# Autodesk Inventor assembly: Linear Actuator 12inch
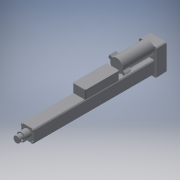
[picture p0: Inventor's stored thumbnail of the model, 180x180]
Saved by Autodesk Inventor 2016 (Build 200138000, 138)
## iProperties
Created: 2018-06-28
Part Number: Linear Actuator 12inch
Document SubType Name: Assembly
Designer: Kade
Author: Kade
## Documents named in this file (3)
- F:\Robotics\Off Season\Blannon\Linear Actuator\Linear Actuator 12inch.iam
- F:\Robotics\Off Season\Blannon\Linear Actuator\Linear Actuator Body.ipt
- F:\Robotics\Off Season\Blannon\Linear Actuator\Linear Actuator Piston.ipt
## Components (2 placed, 2 different names)
1. Linear Actuator Body:1 — Mate:1, Mate:2, Flush:1, Mate:3, Mate:4, Flush:2
2. Linear Actuator Piston:1 — Mate:3, Mate:4, Flush:2
## Relationships (6: Mate 4, Flush 2)
- Mate:1: Linear Actuator Body:1
- Mate:2: Linear Actuator Body:1
- Flush:1: Linear Actuator Body:1
- Mate:3: Linear Actuator Body:1 ↔ Linear Actuator Piston:1
- Mate:4: Linear Actuator Body:1 ↔ Linear Actuator Piston:1
- Flush:2: Linear Actuator Body:1 ↔ Linear Actuator Piston:1
